# Autodesk Inventor assembly: ForearmActuatorShaft
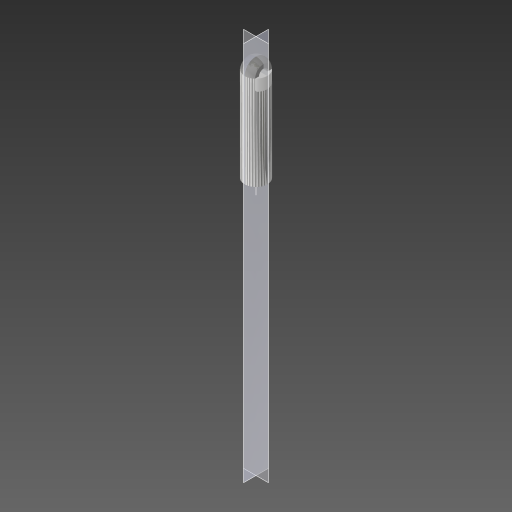
[picture p0: Inventor's stored thumbnail of the model, 512x512]
Saved by Autodesk Inventor 2023 (Build 270158000, 158)
## iProperties
Created: 2023-03-25
Part Number: ForearmActuatorShaft
Document SubType Name: Assembly
Designer: Val
Author: Val
## Documents named in this file (3)
- C:\Users\Val\Desktop\str1ker\parts\external\ForearmActuator\ForearmActuatorShaft.iam
- C:\Users\Val\Desktop\str1ker\parts\external\ForearmActuatorShaft.ipt
- C:\Users\Val\Desktop\str1ker\description\models\src\ForearmActuatorBodyBoundingBox.ipt
## Components (2 placed, 2 different names)
1. ForearmActuatorShaft:1 — Angle:1, Mate:1
2. ForearmActuatorBodyBoundingBox:1 — Flush:1
## Relationships (3: Angle 1, Mate 1, Flush 1)
- Angle:1 (180 deg): ForearmActuatorShaft:1
- Mate:1: ForearmActuatorShaft:1
- Flush:1: ForearmActuatorBodyBoundingBox:1
